# Autodesk Inventor assembly: Assembly mail
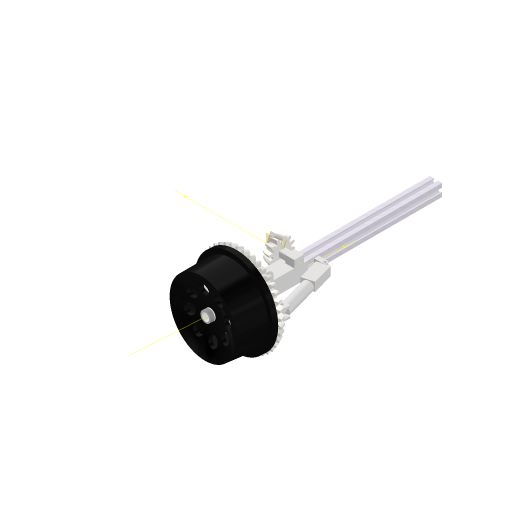
[picture p0: Inventor's stored thumbnail of the model, 512x512]
Saved by Autodesk Inventor 2023 (Build 270158000, 158)
## iProperties
Created: 2023-10-30
Part Number: Assembly mail
Document SubType Name: Assembly
Designer: Juyoung Han
Author: Juyoung Han
## Documents named in this file (11)
- C:\Users\Juyoung Han\Desktop\tankturn\Assembly1.iam
- C:\Users\Juyoung Han\Desktop\tankturn\front axle.ipt
- C:\Users\Juyoung Han\Desktop\Henry 프로젝트\스케치 파일\Nuckle.ipt
- C:\Users\Juyoung Han\Desktop\tankturn\Wheel hub left ver 2.ipt
- C:\Users\Juyoung Han\Desktop\tankturn\HEX HUB ver 1.ipt
- C:\Users\Juyoung Han\Desktop\tankturn\RIM ver 1.ipt
- C:\Users\Juyoung Han\Desktop\tankturn\Bevel Gear12.ipt
- C:\Users\Juyoung Han\Desktop\tankturn\actuator mount 2.ipt
- C:\Users\Juyoung Han\Desktop\tankturn\actuator.ipt
- C:\Users\Juyoung Han\Desktop\tankturn\motor.ipt
- C:\Users\Juyoung Han\Desktop\tankturn\Bevel Gear22.ipt
## Components (10 placed, 10 different names)
1. front axle:1 — Mate:1, Mate:2, Mate:3, Mate:8, Mate:10, Angle:1
2. Nuckle:1 — Mate:1, Mate:2, Rotational:1, Mate:3, Flush:1, Mate:12, Mate:13
3. Wheel hub left ver 2:1 — Rotational:1, Rotational:2, Mate:11
4. HEX HUB ver 1:1 — Rotational:2, Mate:6, Mate:7, Mate:9
5. RIM ver 1:1 — Mate:4, Mate:5, Mate:6, Mate:7, Mate:9
6. Bevel Gear1:1 — Mate:4, Mate:5
7. actuator mount 2:1 — Mate:8, Mate:10, Rotational:3, Angle:1
8. actuator:1 — Rotational:3, Mate:11
9. motor:1 — Flush:1, Mate:12, Mate:13, Rotational:4
10. Bevel Gear2:1 — Rotational:4
## Relationships (19: Mate 13, RevoluteJoint 4, Angle 1, Flush 1)
- Mate:1: front axle:1 ↔ Nuckle:1
- Mate:2: front axle:1 ↔ Nuckle:1
- Rotational:1 [RevoluteJoint]: Nuckle:1 ↔ Wheel hub left ver 2:1
- Mate:3: front axle:1 ↔ Nuckle:1
- Rotational:2 [RevoluteJoint]: Wheel hub left ver 2:1 ↔ HEX HUB ver 1:1
- Mate:4: RIM ver 1:1 ↔ Bevel Gear1:1
- Mate:5: RIM ver 1:1 ↔ Bevel Gear1:1
- Mate:6: HEX HUB ver 1:1 ↔ RIM ver 1:1
- Mate:7: HEX HUB ver 1:1 ↔ RIM ver 1:1
- Mate:8: front axle:1 ↔ actuator mount 2:1
- Mate:9: HEX HUB ver 1:1 ↔ RIM ver 1:1
- Mate:10 (-10.25 mm): front axle:1 ↔ actuator mount 2:1
- Rotational:3 [RevoluteJoint]: actuator mount 2:1 ↔ actuator:1
- Angle:1 (0 deg): front axle:1 ↔ actuator mount 2:1
- Mate:11: Wheel hub left ver 2:1 ↔ actuator:1
- Flush:1: Nuckle:1 ↔ motor:1
- Mate:12: Nuckle:1 ↔ motor:1
- Mate:13 (45 mm): Nuckle:1 ↔ motor:1
- Rotational:4 [RevoluteJoint]: motor:1 ↔ Bevel Gear2:1
